# Autodesk Inventor assembly: sim_cyc_nema17
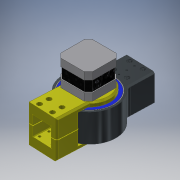
[picture p0: Inventor's stored thumbnail of the model, 180x180]
Saved by Autodesk Inventor 2017 (Build 210142000, 142)
## iProperties
Created: 2021-02-24
Part Number: sim_cyc_nema17
Document SubType Name: Assembly
Designer: paulg
Author: paulg
## Documents named in this file (27)
- C:\play\3D_play\simple_cyc_nema17\sim_cyc_nema17.iam
- C:\play\3D_play\simple_cyc_nema17\ecc_shaft.ipt
- C:\play\3D_play\Cycloid CAD\65x50x7 bearing.ipt
- C:\play\3D_play\robot arm\Motor_paso.ipt
- C:\play\3D_play\simple_cyc_nema17\base_stepper.ipt
- C:\play\3D_play\simple_cyc_nema17\output_housing.ipt
- C:\play\3D_play\Cycloid CAD\18x12x4 bearing.ipt
- C:\play\3D_play\bldc_capstan\27x20x4 bearing.ipt
- C:\play\3D_play\simple_cyc_nema17\base_top.ipt
- C:\play\3D_play\simple_cyc_nema17\Main_equation_step_simple.ipt
- C:\play\3D_play\simple_cyc_nema17\Main_equation_step_simple_upper.ipt
- C:\play\3D_play\simple_cyc_nema17\bottom_clip.ipt
- C:\play\3D_play\simple_cyc_nema17\top_clip.ipt
- C:\play\3D_play\simple_cyc_nema17\m3 nut.ipt
- C:\play\3D_play\simple_cyc_nema17\m3_setscrew.ipt
- C:\play\3D_play\Cycloid CAD\15x10x4 bearing.ipt
- C:\play\3D_play\Cycloid CAD\mag_6mm.iam
- C:\play\3D_play\old-new-cycloidal\foc.ipt
- C:\play\3D_play\old-new-cycloidal\dan2.ipt
- C:\play\3D_play\old-new-cycloidal\Mike2.ipt
- C:\play\3D_play\old-new-cycloidal\Matt.ipt
- C:\play\3D_play\old-new-cycloidal\Tim.ipt
- C:\play\encoder\PCB\ENCODER_AS_MA.iam
- C:\play\3D_play\Cycloid CAD\8x5x2.5 bearing.ipt
- C:\play\3D_play\old-new-cycloidal\3mm_pin.ipt
- C:\play\3D_play\simple_cyc_nema17\joint mag.ipt
- C:\play\3D_play\old-new-cycloidal\Parameters_stepper_simple.xlsx
## Components (52 placed, 25 different names)
1. ecc_shaft:1 — Insert:5, Insert:7, Insert:8, Mate:2, Insert:14, Mate:3, Insert:16, Insert:17, Insert:18, Insert:21, Insert:29, Insert:47
2. 65x50x7 bearing:1 — Insert:2, Insert:48
3. Motor_paso:1 — Mate:1, Insert:47
4. base_stepper:1 — Mate:1, Insert:2, Flush:1, Insert:39, Insert:40, Insert:41, Insert:42, Insert:43, Insert:44, Insert:45, Insert:46
5. output_housing:1 — Insert:9, Insert:48, Insert:49, Mate:7
6. 18x12x4 bearing:1 — Insert:8, Insert:12
7. 18x12x4 bearing:2 — Insert:7
8. 27x20x4 bearing:1 — Insert:5
9. 27x20x4 bearing:2 — Insert:20, Insert:29
10. base_top:1 — Insert:10, Flush:1, Mate:4, Mate:5, Mate:6
11. 65x50x7 bearing:2 — Insert:9, Insert:10
12. Main_equation_step_simple_upper:1 — Insert:12, Insert:31, Insert:32, Insert:33, Insert:34, Insert:35, Insert:36, Insert:37, Insert:38
13. bottom_clip:1 — Mate:2, Insert:14
14. top_clip:1 — Mate:3, Insert:16, Insert:19
15. m3 nut:1 — Insert:17
16. m3_setscrew:1 — Insert:18
17. 15x10x4 bearing:1 — Insert:19
18. Main_equation_step_simple:1 — Insert:20, Insert:22, Insert:23, Insert:24, Insert:25, Insert:26, Insert:27, Insert:28, Insert:30
19. mag_6mm:1 [sub-assembly] — Insert:21
20. foc:1
21. dan2:1
22. Mike2:1
23. Matt:1
24. Tim:1
25. ENCODER_AS_MA:1 [sub-assembly] — Mate:4, Mate:5, Mate:6, Insert:51
26. 8x5x2.5 bearing:1 — Insert:22
27. 8x5x2.5 bearing:2 — Insert:36
28. 8x5x2.5 bearing:3 — Insert:35
29. 8x5x2.5 bearing:4 — Insert:34, Tangent:1
30. 8x5x2.5 bearing:5 — Insert:32
31. 8x5x2.5 bearing:6 — Insert:30, Tangent:2
32. 8x5x2.5 bearing:7 — Insert:31
33. 8x5x2.5 bearing:8 — Insert:23
34. 8x5x2.5 bearing:9 — Insert:24
35. 8x5x2.5 bearing:10 — Insert:25
36. 8x5x2.5 bearing:11 — Insert:28
37. 8x5x2.5 bearing:12 — Insert:37
38. 8x5x2.5 bearing:14 — Insert:33
39. 8x5x2.5 bearing:19 — Insert:27
40. 8x5x2.5 bearing:20 — Insert:26
41. 8x5x2.5 bearing:21 — Insert:38
42. 3mm_pin:2 — Insert:41
43. 3mm_pin:4 — Insert:46, Tangent:1, Tangent:2
44. 3mm_pin:5 — Insert:44
45. 3mm_pin:6 — Insert:42
46. 3mm_pin:7 — Insert:39
47. 3mm_pin:8 — Insert:40
48. 3mm_pin:9 — Insert:45
49. 3mm_pin:10 — Insert:43
50. joint mag:1 — Insert:49, Mate:7, Insert:50
51. mag_6mm:2 [sub-assembly] — Insert:50
52. ENCODER_AS_MA:2 [sub-assembly] — Insert:51
## Relationships (54: Insert 44, Mate 7, Tangent 2, Flush 1)
- Mate:1: Motor_paso:1 ↔ base_stepper:1
- Insert:2: 65x50x7 bearing:1 ↔ base_stepper:1
- Insert:5: ecc_shaft:1 ↔ 27x20x4 bearing:1
- Insert:7: ecc_shaft:1 ↔ 18x12x4 bearing:2
- Insert:8: ecc_shaft:1 ↔ 18x12x4 bearing:1
- Insert:9: output_housing:1 ↔ 65x50x7 bearing:2
- Insert:10: base_top:1 ↔ 65x50x7 bearing:2
- Flush:1: base_stepper:1 ↔ base_top:1
- Insert:12: 18x12x4 bearing:1 ↔ Main_equation_step_simple_upper:1
- Mate:2: ecc_shaft:1 ↔ bottom_clip:1
- Insert:14: ecc_shaft:1 ↔ bottom_clip:1
- Mate:3: ecc_shaft:1 ↔ top_clip:1
- Insert:16: ecc_shaft:1 ↔ top_clip:1
- Insert:17: ecc_shaft:1 ↔ m3 nut:1
- Insert:18 (-3 mm): ecc_shaft:1 ↔ m3_setscrew:1
- Insert:19: top_clip:1 ↔ 15x10x4 bearing:1
- Insert:20: 27x20x4 bearing:2 ↔ Main_equation_step_simple:1
- Insert:21: ecc_shaft:1 ↔ mag_6mm:1
- Mate:4: base_top:1 ↔ ENCODER_AS_MA:1
- Mate:5 (0.5 mm): base_top:1 ↔ ENCODER_AS_MA:1
- Mate:6 (0.5 mm): base_top:1 ↔ ENCODER_AS_MA:1
- Insert:22: Main_equation_step_simple:1 ↔ 8x5x2.5 bearing:1
- Insert:23: Main_equation_step_simple:1 ↔ 8x5x2.5 bearing:8
- Insert:24: Main_equation_step_simple:1 ↔ 8x5x2.5 bearing:9
- Insert:25: Main_equation_step_simple:1 ↔ 8x5x2.5 bearing:10
- Insert:26: Main_equation_step_simple:1 ↔ 8x5x2.5 bearing:20
- Insert:27: Main_equation_step_simple:1 ↔ 8x5x2.5 bearing:19
- Insert:28: Main_equation_step_simple:1 ↔ 8x5x2.5 bearing:11
- Insert:29: ecc_shaft:1 ↔ 27x20x4 bearing:2
- Insert:30: Main_equation_step_simple:1 ↔ 8x5x2.5 bearing:6
- Insert:31: Main_equation_step_simple_upper:1 ↔ 8x5x2.5 bearing:7
- Insert:32: Main_equation_step_simple_upper:1 ↔ 8x5x2.5 bearing:5
- Insert:33: Main_equation_step_simple_upper:1 ↔ 8x5x2.5 bearing:14
- Insert:34: Main_equation_step_simple_upper:1 ↔ 8x5x2.5 bearing:4
- Insert:35: Main_equation_step_simple_upper:1 ↔ 8x5x2.5 bearing:3
- Insert:36: Main_equation_step_simple_upper:1 ↔ 8x5x2.5 bearing:2
- Insert:37: Main_equation_step_simple_upper:1 ↔ 8x5x2.5 bearing:12
- Insert:38: Main_equation_step_simple_upper:1 ↔ 8x5x2.5 bearing:21
- Insert:39: base_stepper:1 ↔ 3mm_pin:7
- Insert:40: base_stepper:1 ↔ 3mm_pin:8
- Insert:41: base_stepper:1 ↔ 3mm_pin:2
- Insert:42: base_stepper:1 ↔ 3mm_pin:6
- Insert:43: base_stepper:1 ↔ 3mm_pin:10
- Insert:44: base_stepper:1 ↔ 3mm_pin:5
- Insert:45: base_stepper:1 ↔ 3mm_pin:9
- Insert:46: base_stepper:1 ↔ 3mm_pin:4
- Insert:47 (1 mm): ecc_shaft:1 ↔ Motor_paso:1
- Tangent:1: 8x5x2.5 bearing:4 ↔ 3mm_pin:4
- Tangent:2: 8x5x2.5 bearing:6 ↔ 3mm_pin:4
- Insert:48: 65x50x7 bearing:1 ↔ output_housing:1
- Insert:49: output_housing:1 ↔ joint mag:1
- Mate:7: output_housing:1 ↔ joint mag:1
- Insert:50 (0.5 mm): joint mag:1 ↔ mag_6mm:2
- Insert:51 (4 mm): ENCODER_AS_MA:1 ↔ ENCODER_AS_MA:2
## Named parameters: N_ = 25, E_ = 1 mm, Rr_ = 2 mm, R_ = 31.5 mm
